# Autodesk Inventor assembly: 742a 2.1 Catapult
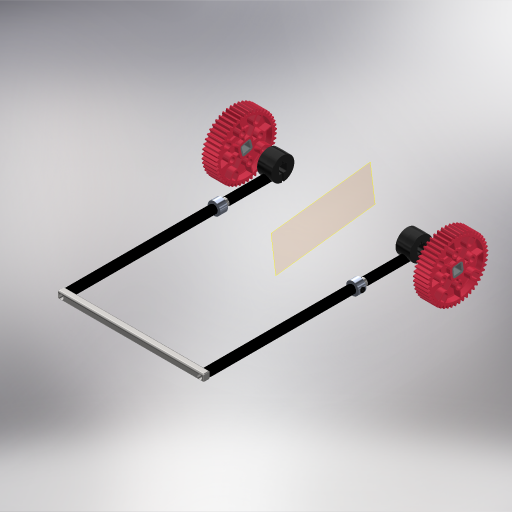
[picture p0: Inventor's stored thumbnail of the model, 512x512]
Saved by Autodesk Inventor 2024 (Build 280153000, 153)
## iProperties
Created: 2023-10-21
Part Number: 742a 2.1 Catapult
Document SubType Name: Assembly
Designer: aaron
Author: aaron
## Documents named in this file (9)
- X:\VexU Github\PERRY-15-\Perry VEXU\Library\Subsystems\15 2.0 Catapult.iam
- X:\VexU Github\PERRY-15-\Perry VEXU\Library\VEX Library\Motion\HS Shaft\HS Shaft Collar.ipt
- C:\Users\aaron\Documents\Inventor\TritonRobotics\library\VEX Library\Structure\Standoff.ipt
- X:\VexU Github\PERRY-15-\Perry VEXU\Library\VEX Library\Motion\Gears\High Strength\48 Tooth\48 High Strength Gear V2.ipt
- X:\VexU Github\PERRY-15-\Perry VEXU\Library\VEX Library\Structure\Standoff\Standoff 1.5.ipt
- X:\VexU Github\PERRY-15-\Perry VEXU\Library\VEX Library\Structure\Metal Spacers\.125 .25 OD.ipt
- X:\VexU Github\PERRY-15-\Perry VEXU\Library\VEX Library\Motion\Shaft Collar with Set Screw.ipt
- X:\VexU Github\PERRY-15-\Perry VEXU\Library\VEX Library\Structure\Standoff\Standoff 5.ipt
- X:\VexU Github\PERRY-15-\Perry VEXU\Library\VEX Library\Structure\hs shaft\cata Beam.ipt
## Components (13 placed, 7 different names)
1. HS Shaft Collar:1 — Mate:1, Mate:6, Mate:15, Mate:16, Mate:47
2. HS Shaft Collar:2 — Mate:1, Mate:7, Mate:14, Mate:17, Mate:46
3. 48 High Strength Gear V2:1 — Mate:6, Mate:47
4. 48 High Strength Gear V2:2 — Mate:7, Mate:46
5. Standoff 1.5:1 — Mate:15, Mate:16, Mate:25, Mate:26, Mate:27
6. Standoff 1.5:2 — Mate:14, Mate:17, Mate:23, Mate:24
7. .125 .25 OD:1 — Mate:25, Mate:26
8. .125 .25 OD:2 — Mate:23, Mate:24, Mate:33
9. Shaft Collar with Set Screw:1 — Mate:27, Mate:40, Mate:41
10. Shaft Collar with Set Screw:2 — Mate:33, Mate:39, Mate:42
11. Standoff 5:5 — Mate:39, Mate:42, Mate:43
12. Standoff 5:6 — Mate:40, Mate:41, Mate:44, Mate:45
13. cata Beam:1 — Mate:43, Mate:44, Mate:45
## Relationships (22: Mate 22)
- Mate:1: HS Shaft Collar:1 ↔ HS Shaft Collar:2
- Mate:6: HS Shaft Collar:1 ↔ 48 High Strength Gear V2:1
- Mate:7: HS Shaft Collar:2 ↔ 48 High Strength Gear V2:2
- Mate:14: HS Shaft Collar:2 ↔ Standoff 1.5:2
- Mate:15: HS Shaft Collar:1 ↔ Standoff 1.5:1
- Mate:16: HS Shaft Collar:1 ↔ Standoff 1.5:1
- Mate:17: HS Shaft Collar:2 ↔ Standoff 1.5:2
- Mate:23: Standoff 1.5:2 ↔ .125 .25 OD:2
- Mate:24: Standoff 1.5:2 ↔ .125 .25 OD:2
- Mate:25: Standoff 1.5:1 ↔ .125 .25 OD:1
- Mate:26: Standoff 1.5:1 ↔ .125 .25 OD:1
- Mate:27: Standoff 1.5:1 ↔ Shaft Collar with Set Screw:1
- Mate:33: .125 .25 OD:2 ↔ Shaft Collar with Set Screw:2
- Mate:39: Shaft Collar with Set Screw:2 ↔ Standoff 5:5
- Mate:40: Shaft Collar with Set Screw:1 ↔ Standoff 5:6
- Mate:41: Shaft Collar with Set Screw:1 ↔ Standoff 5:6
- Mate:42: Shaft Collar with Set Screw:2 ↔ Standoff 5:5
- Mate:43: Standoff 5:5 ↔ cata Beam:1
- Mate:44: Standoff 5:6 ↔ cata Beam:1
- Mate:45: Standoff 5:6 ↔ cata Beam:1
- Mate:46 (19.05 mm): HS Shaft Collar:2 ↔ 48 High Strength Gear V2:2
- Mate:47 (19.05 mm): HS Shaft Collar:1 ↔ 48 High Strength Gear V2:1
